# Autodesk Inventor assembly: Crank_Fixation
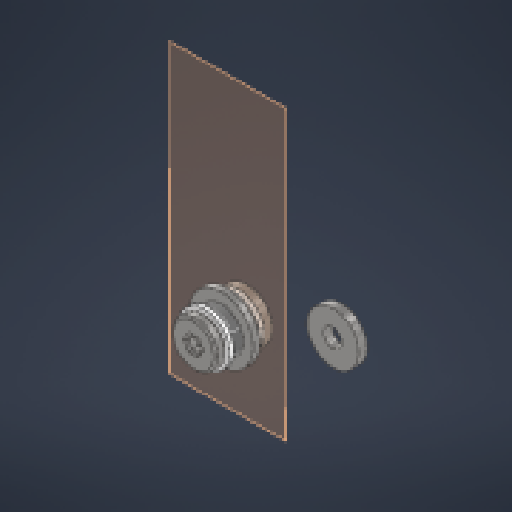
[picture p0: Inventor's stored thumbnail of the model, 512x512]
Saved by Autodesk Inventor 2024.3 (Build 283343000, 343)
## iProperties
Created: 2025-01-10
Part Number: Crank_Fixation
Document SubType Name: Assembly
Designer: ASUS
Author: ASUS
## Documents named in this file (6)
- C:\Users\ASUS\Desktop\Anti_Backlash_Structure_OP\v4_Frame_2025\ALI\Crank_Fixation.iam
- C:\Users\ASUS\Desktop\Anti_Backlash_Structure_OP\v4_Frame_2025\ALI\M5-D6-8mm.ipt
- C:\Users\ASUS\Desktop\Anti_Backlash_Structure_OP\MISUMI\LED-0606.ipt
- C:\Users\ASUS\Desktop\Anti_Backlash_Structure_OP\MISUMI\TT-0612-101.ipt
- C:\Users\ASUS\Desktop\Anti_Backlash_Structure_OP\V2_Frame(2025)\Ubber_Washer_1.5mm.ipt
- C:\Users\ASUS\Desktop\Anti_Backlash_Structure_OP\MISUMI\C-WSSA12-5-2.ipt
## Components (6 placed, 5 different names)
1. LED-0606:1
2. TT-0612-10:1 — 삽입:5
3. TT-0612-10:2 — 삽입:6
4. Ubber_Washer_1.5mm:1
5. M5-D6-8mm:1 — 삽입:5
6. C-WSSA12-5-2:1 — 삽입:6
## Relationships (5: Insert 5)
- [Insert]: LED-0606:1 ↔ TT-0612-10:1
- [Insert]: LED-0606:1 ↔ TT-0612-10:2
- [Insert]: LED-0606:1 ↔ Ubber_Washer_1.5mm:1
- 삽입:5 [Insert]: TT-0612-10:1 ↔ M5-D6-8mm:1
- 삽입:6 [Insert]: TT-0612-10:2 ↔ C-WSSA12-5-2:1
